# Autodesk Inventor assembly: BG_Mittelkonsole
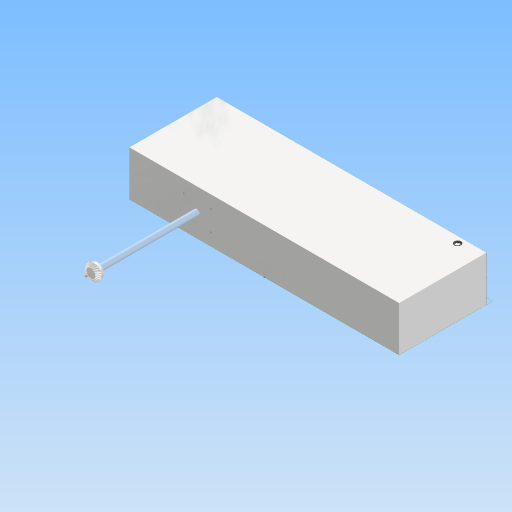
[picture p0: Inventor's stored thumbnail of the model, 512x512]
Saved by Autodesk Inventor 2024.4 (Build 284460000, 460)
## iProperties
Created: 2026-01-19
Part Number: BG_Mittelkonsole
Document SubType Name: Assembly
Designer: windows-desktop
Mass: 21086 g
Surface Area: 40250.2 cm^2
Volume: 17591.1 cm^3
Density: 1.19868 g/cm^3
## Documents named in this file (14)
- C:\Users\windows-desktop\Desktop\Studium\Konstruktion\VaultWorkspace\Daten\I60-Konstruktion\I60-Gruppe-4\Bluhm\Daten\I60-Konstruktion\I60-Gruppe-4\Bluhm\Deck_Getriebe\BG_Mittelkonsole.iam
- C:\Users\windows-desktop\Desktop\Studium\Konstruktion\VaultWorkspace\Daten\I60-Konstruktion\I60-Gruppe-4\Bluhm\Daten\I60-Konstruktion\I60-Gruppe-4\Bluhm\Deck_Getriebe\Wellennut.ipt
- C:\Users\windows-desktop\Desktop\Studium\Konstruktion\VaultWorkspace\Daten\I60-Konstruktion\I60-Gruppe-4\Bluhm\Normteile\de-DE\DIN 3760 A\DIN 3760 - A - 20 x 30 x 7 - NBR.ipt
- C:\Users\windows-desktop\Desktop\Studium\Konstruktion\VaultWorkspace\Daten\I60-Konstruktion\I60-Gruppe-4\Bluhm\Normteile\de-DE\DIN 625 SKF(3)\DIN 625 SKF - SKF (61807-RZ).ipt
- C:\Users\windows-desktop\Desktop\Studium\Konstruktion\VaultWorkspace\Daten\I60-Konstruktion\I60-Gruppe-4\Bluhm\Normteile\de-DE\DIN 625 SKF(3)\DIN 625 SKF - SKF (61804-RZ).ipt
- C:\Users\windows-desktop\Desktop\Studium\Konstruktion\VaultWorkspace\Daten\I60-Konstruktion\I60-Gruppe-4\Bluhm\Normteile\de-DE\DIN 625 SKF(3)\DIN 625 SKF - SKF (61912-RZ).ipt
- C:\Users\windows-desktop\Desktop\Studium\Konstruktion\VaultWorkspace\Daten\I60-Konstruktion\I60-Gruppe-4\Bluhm\Daten\I60-Konstruktion\I60-Gruppe-4\Bluhm\Verbindung_Deck_Antrieb\Kegelrad_20x10_01.ipt
- C:\Users\windows-desktop\Desktop\Studium\Konstruktion\VaultWorkspace\Daten\I60-Konstruktion\I60-Gruppe-4\Bluhm\Daten\I60-Konstruktion\I60-Gruppe-4\Bluhm\Verbindung_Deck_Antrieb\Welle.ipt
- C:\Users\windows-desktop\Desktop\Studium\Konstruktion\VaultWorkspace\Daten\I60-Konstruktion\I60-Gruppe-4\Bluhm\Daten\I60-Konstruktion\I60-Gruppe-4\Bluhm\Verbindung_Deck_Antrieb\Wellennut_Verbindung_Deck_Antrieb.ipt
- C:\Users\windows-desktop\Desktop\Studium\Konstruktion\VaultWorkspace\Daten\I60-Konstruktion\I60-Gruppe-4\Bluhm\Daten\I60-Konstruktion\I60-Gruppe-4\Bluhm\Verbindung_Deck_Antrieb\Kegelrad_20x10_02.ipt
- C:\Users\windows-desktop\Desktop\Studium\Konstruktion\VaultWorkspace\Daten\I60-Konstruktion\I60-Gruppe-4\Bluhm\Daten\I60-Konstruktion\I60-Gruppe-4\Bluhm\Deck_Getriebe\Neu Kegelrad_Version01.ipt
- C:\Users\windows-desktop\Desktop\Studium\Konstruktion\VaultWorkspace\Daten\I60-Konstruktion\I60-Gruppe-4\Bluhm\Daten\I60-Konstruktion\I60-Gruppe-4\Bluhm\Deck_Getriebe\Neu Kegelrad_Version02.ipt
- C:\Users\windows-desktop\Desktop\Studium\Konstruktion\VaultWorkspace\Daten\I60-Konstruktion\I60-Gruppe-4\Bluhm\Daten\I60-Konstruktion\I60-Gruppe-4\Bluhm\Deck_Getriebe\Welle_Deck_Getriebe.ipt
- C:\Users\windows-desktop\Desktop\Studium\Konstruktion\VaultWorkspace\Daten\I60-Konstruktion\I60-Gruppe-4\Bluhm\Daten\I60-Konstruktion\I60-Gruppe-4\Bluhm\Deck_Getriebe\Mittelkonsole.ipt
## Components (20 placed, 11 different names)
1. DIN 3760 A A - 20 x 30 x 7 - NBR:1 — Einfügen:21
2. DIN 3760 A A - 20 x 30 x 7 - NBR:2 — Einfügen:22
3. DIN 625 SKF- mit Dichtung mit niedriger Reibung, einseitig abgedichtet SKF (61807-RZ):1 — Einfügen:25
4. DIN 625 SKF- mit Dichtung mit niedriger Reibung, einseitig abgedichtet SKF (61807-RZ):2 — Einfügen:26
5. DIN 625 SKF- mit Dichtung mit niedriger Reibung, einseitig abgedichtet SKF (61804-RZ):2 — Einfügen:24
6. DIN 625 SKF- mit Dichtung mit niedriger Reibung, einseitig abgedichtet SKF (61804-RZ):3 — Einfügen:23
7. Wellennut:1 — Fluchtend:8, Passend:20, Fluchtend:10, Passend:24
8. Kegelrad1:7 — Einfügen:19, Fluchtend:5, Fluchtend:6, Passend:16, Passend:17
9. DIN 625 SKF- mit Dichtung mit niedriger Reibung, einseitig abgedichtet SKF (61912-RZ):2 — Einfügen:19, Einfügen:27
10. Welle:1 — Fluchtend:3, Fluchtend:4, Passend:12, Passend:13, Passend:14, Passend:15
11. Wellennut_Verbindung_Deck_Antrieb:1 — Fluchtend:4, Passend:12, Passend:13, Fluchtend:7, Passend:18, Passend:19
12. Wellennut_Verbindung_Deck_Antrieb:2 — Fluchtend:3, Passend:14, Passend:15, Fluchtend:5, Fluchtend:6, Passend:16, Passend:17
13. Kegelrad2:7 — Fluchtend:7, Passend:18, Passend:19
14. Kegelrad1:8 — Fluchtend:12, Passend:27, Passend:28, Einfügen:28
15. Kegelrad2:8 — Fluchtend:10, Passend:24, Einfügen:20
16. Welle_Deck_Getriebe:1 — Fluchtend:8, Passend:20, Einfügen:20, Fluchtend:11, Passend:25, Passend:26
17. Wellennut:3 — Fluchtend:11, Passend:25, Passend:26, Fluchtend:12, Passend:27, Passend:28
18. Kegelrad2:9 — Einfügen:30
19. Kegelrad2:10 — Einfügen:29
20. Mittelkonsole:1 — Einfügen:21, Einfügen:22, Einfügen:23, Einfügen:24, Einfügen:25, Einfügen:26, Einfügen:27, Einfügen:28, Einfügen:29, Einfügen:30
## Relationships (35: Mate 14, Insert 12, Flush 9)
- Einfügen:19 [Insert]: Kegelrad1:7 ↔ DIN 625 SKF- mit Dichtung mit niedriger Reibung, einseitig abgedichtet SKF (61912-RZ):2
- Fluchtend:3 [Flush]: Welle:1 ↔ Wellennut_Verbindung_Deck_Antrieb:2
- Fluchtend:4 [Flush]: Welle:1 ↔ Wellennut_Verbindung_Deck_Antrieb:1
- Passend:12 [Mate]: Welle:1 ↔ Wellennut_Verbindung_Deck_Antrieb:1
- Passend:13 [Mate]: Welle:1 ↔ Wellennut_Verbindung_Deck_Antrieb:1
- Passend:14 [Mate]: Welle:1 ↔ Wellennut_Verbindung_Deck_Antrieb:2
- Passend:15 [Mate]: Welle:1 ↔ Wellennut_Verbindung_Deck_Antrieb:2
- Fluchtend:5 [Flush]: Kegelrad1:7 ↔ Wellennut_Verbindung_Deck_Antrieb:2
- Fluchtend:6 [Flush]: Kegelrad1:7 ↔ Wellennut_Verbindung_Deck_Antrieb:2
- Passend:16 [Mate]: Kegelrad1:7 ↔ Wellennut_Verbindung_Deck_Antrieb:2
- Passend:17 [Mate]: Kegelrad1:7 ↔ Wellennut_Verbindung_Deck_Antrieb:2
- Fluchtend:7 [Flush]: Wellennut_Verbindung_Deck_Antrieb:1 ↔ Kegelrad2:7
- Passend:18 [Mate]: Wellennut_Verbindung_Deck_Antrieb:1 ↔ Kegelrad2:7
- Passend:19 [Mate]: Wellennut_Verbindung_Deck_Antrieb:1 ↔ Kegelrad2:7
- Fluchtend:8 [Flush]: Wellennut:1 ↔ Welle_Deck_Getriebe:1
- Passend:20 [Mate]: Wellennut:1 ↔ Welle_Deck_Getriebe:1
- Fluchtend:10 [Flush]: Wellennut:1 ↔ Kegelrad2:8
- Passend:24 [Mate]: Wellennut:1 ↔ Kegelrad2:8
- Einfügen:20 [Insert]: Kegelrad2:8 ↔ Welle_Deck_Getriebe:1
- Fluchtend:11 [Flush]: Welle_Deck_Getriebe:1 ↔ Wellennut:3
- Passend:25 [Mate]: Welle_Deck_Getriebe:1 ↔ Wellennut:3
- Passend:26 [Mate]: Welle_Deck_Getriebe:1 ↔ Wellennut:3
- Fluchtend:12 [Flush]: Kegelrad1:8 ↔ Wellennut:3
- Passend:27 [Mate]: Kegelrad1:8 ↔ Wellennut:3
- Passend:28 [Mate]: Kegelrad1:8 ↔ Wellennut:3
- Einfügen:21 [Insert]: DIN 3760 A A - 20 x 30 x 7 - NBR:1 ↔ Mittelkonsole:1
- Einfügen:22 [Insert]: DIN 3760 A A - 20 x 30 x 7 - NBR:2 ↔ Mittelkonsole:1
- Einfügen:23 [Insert]: DIN 625 SKF- mit Dichtung mit niedriger Reibung, einseitig abgedichtet SKF (61804-RZ):3 ↔ Mittelkonsole:1
- Einfügen:24 [Insert]: DIN 625 SKF- mit Dichtung mit niedriger Reibung, einseitig abgedichtet SKF (61804-RZ):2 ↔ Mittelkonsole:1
- Einfügen:25 [Insert]: DIN 625 SKF- mit Dichtung mit niedriger Reibung, einseitig abgedichtet SKF (61807-RZ):1 ↔ Mittelkonsole:1
- Einfügen:26 [Insert]: DIN 625 SKF- mit Dichtung mit niedriger Reibung, einseitig abgedichtet SKF (61807-RZ):2 ↔ Mittelkonsole:1
- Einfügen:27 [Insert]: DIN 625 SKF- mit Dichtung mit niedriger Reibung, einseitig abgedichtet SKF (61912-RZ):2 ↔ Mittelkonsole:1
- Einfügen:28 [Insert]: Kegelrad1:8 ↔ Mittelkonsole:1
- Einfügen:29 [Insert]: Kegelrad2:10 ↔ Mittelkonsole:1
- Einfügen:30 [Insert]: Kegelrad2:9 ↔ Mittelkonsole:1
